# Autodesk Inventor assembly: DoorLock
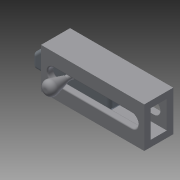
[picture p0: Inventor's stored thumbnail of the model, 180x180]
Saved by Autodesk Inventor 2015 (Build 190159000, 159)
## iProperties
Created: 2015-04-07
Part Number: DoorLock
Document SubType Name: Assembly
Designer: WASHHSST
Author: WASHHSST
## Documents named in this file (4)
- C:\Users\washhsst\Documents\GitHub\myWork\DoorLock.iam
- C:\Users\washhsst\Documents\GitHub\myWork\OmniDoorLock\bolt.ipt
- C:\Users\washhsst\Documents\GitHub\myWork\OmniDoorLock\housing.ipt
- C:\Users\washhsst\Documents\GitHub\myWork\OmniDoorLock\peg.ipt
## Components (3 placed, 3 different names)
1. bolt:1 — Insert:1, Mate:1, Mate:2, Mate:3, Mate:4
2. housing:1 — Mate:1, Mate:2, Mate:3, Mate:4, Mate:5, Mate:6
3. peg:1 — Insert:1, Mate:5, Mate:6
## Relationships (7: Mate 6, Insert 1)
- Insert:1: bolt:1 ↔ peg:1
- Mate:1: bolt:1 ↔ housing:1
- Mate:2: bolt:1 ↔ housing:1
- Mate:3: bolt:1 ↔ housing:1
- Mate:4: bolt:1 ↔ housing:1
- Mate:5: housing:1 ↔ peg:1
- Mate:6: housing:1 ↔ peg:1
